# Autodesk Inventor assembly: SimpleBot
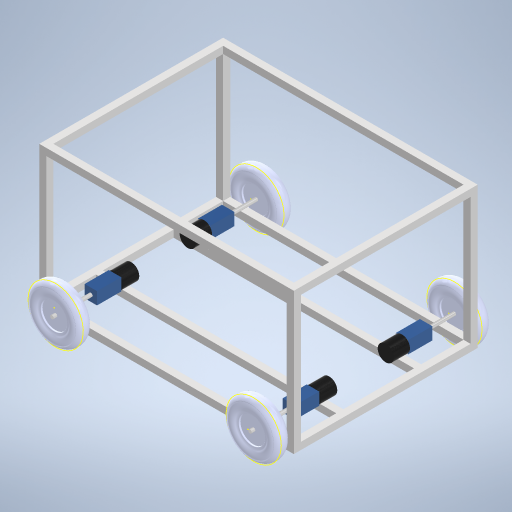
[picture p0: Inventor's stored thumbnail of the model, 512x512]
Saved by Autodesk Inventor 2023 (Build 270158000, 158)
## iProperties
Created: 2022-08-31
Part Number: SimpleBot
Document SubType Name: Assembly
Designer: PC
Author: PC
## Documents named in this file (4)
- C:\Users\PC\Documents\PersonalCAD\ARCIGVC\GazeboTesting\SimpleBox1\SimpleBot.iam
- C:\Users\PC\Documents\PersonalCAD\ARCIGVC\GazeboTesting\SimpleBox1\Chassis.ipt
- C:\Users\PC\Documents\PersonalCAD\ARCIGVC\GazeboTesting\SimpleBox1\MotorAxel.ipt
- C:\Users\PC\Documents\PersonalCAD\ARCIGVC\Pullman's Example\Pneumatic Wheel 8in.ipt
## Components (9 placed, 3 different names)
1. Chassis:1 — Mate:1, Flush:1, Mate:3, Mate:4, Mate:5, Mate:6, Flush:3, Flush:4, Flush:5, Mate:7, Mate:8, Mate:9
2. MotorAxel:1 — Mate:5, Flush:5, Mate:7, Mate:11, Flush:7
3. MotorAxel:2 — Mate:1, Flush:1, Mate:2, Flush:2, Mate:3
4. MotorAxel:3 — Mate:4, Flush:4, Mate:8, Mate:12, Flush:6
5. MotorAxel:4 — Mate:6, Flush:3, Mate:9, Mate:10, Flush:8
6. Pneumatic Wheel 8in:1 — Mate:2, Flush:2
7. Pneumatic Wheel 8in:2 — Mate:12, Flush:6
8. Pneumatic Wheel 8in:3 — Mate:11, Flush:7
9. Pneumatic Wheel 8in:4 — Mate:10, Flush:8
## Relationships (20: Mate 12, Flush 8)
- Mate:1: Chassis:1 ↔ MotorAxel:2
- Flush:1 (-25.4 mm): Chassis:1 ↔ MotorAxel:2
- Mate:2: MotorAxel:2 ↔ Pneumatic Wheel 8in:1
- Flush:2 (-12.7 mm): MotorAxel:2 ↔ Pneumatic Wheel 8in:1
- Mate:3 (53.975 mm): Chassis:1 ↔ MotorAxel:2
- Mate:4: Chassis:1 ↔ MotorAxel:3
- Mate:5: Chassis:1 ↔ MotorAxel:1
- Mate:6: Chassis:1 ↔ MotorAxel:4
- Flush:3 (-25.4 mm): Chassis:1 ↔ MotorAxel:4
- Flush:4 (-25.4 mm): Chassis:1 ↔ MotorAxel:3
- Flush:5 (-25.4 mm): Chassis:1 ↔ MotorAxel:1
- Mate:7 (53.975 mm): Chassis:1 ↔ MotorAxel:1
- Mate:8 (53.975 mm): Chassis:1 ↔ MotorAxel:3
- Mate:9 (53.975 mm): Chassis:1 ↔ MotorAxel:4
- Mate:10: MotorAxel:4 ↔ Pneumatic Wheel 8in:4
- Mate:11: MotorAxel:1 ↔ Pneumatic Wheel 8in:3
- Mate:12: MotorAxel:3 ↔ Pneumatic Wheel 8in:2
- Flush:6 (-12.7 mm): MotorAxel:3 ↔ Pneumatic Wheel 8in:2
- Flush:7 (12.7 mm): MotorAxel:1 ↔ Pneumatic Wheel 8in:3
- Flush:8 (-12.7 mm): MotorAxel:4 ↔ Pneumatic Wheel 8in:4
